# Autodesk Inventor assembly: Assembly1
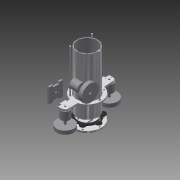
[picture p0: Inventor's stored thumbnail of the model, 180x180]
Saved by Autodesk Inventor 2015 (Build 190159000, 159)
## iProperties
Created: 2015-02-28
Part Number: Assembly1
Document SubType Name: Assembly
Designer: Qiuyang
Author: Qiuyang
## Documents named in this file (8)
- C:\Users\Qiuyang\Dropbox\VIP\SeaPerch\Dimensions\Aluminium_structure\Assembly1.iam
- C:\Users\Qiuyang\Dropbox\VIP\SeaPerch\Dimensions\Aluminium_structure\tube.ipt
- C:\Users\Qiuyang\Dropbox\VIP\SeaPerch\Dimensions\Aluminium_structure\rubber ring.ipt
- C:\Users\Qiuyang\Dropbox\VIP\SeaPerch\Dimensions\Aluminium_structure\threaded rod.ipt
- C:\Users\Qiuyang\Dropbox\VIP\SeaPerch\Dimensions\Aluminium_structure\cap with wire cut.ipt
- C:\Users\Qiuyang\Dropbox\VIP\SeaPerch\Dimensions\Aluminium_structure\middle plate.ipt
- C:\Users\Qiuyang\Dropbox\VIP\SeaPerch\Dimensions\Aluminium_structure\motor.ipt
- C:\Users\Qiuyang\Dropbox\VIP\SeaPerch\Dimensions\Aluminium_structure\motor holder.ipt
## Components (12 placed, 7 different names)
1. tube:1 — Insert:1, Insert:6, Insert:7
2. threaded rod:1 — Insert:5
3. threaded rod:2 — Insert:4
4. threaded rod:3 — Insert:3
5. rubber ring:1 — Insert:1, Insert:3, Insert:4, Insert:5
6. cap with wire cut:1 — Insert:6
7. middle plate:1 — Insert:7, Insert:8, Insert:9, Insert:10, Insert:11
8. motor:1 — Insert:8, Insert:11
9. motor:2 — Insert:9, Insert:10
10. motor:3
11. motor holder:1
12. motor holder:2
## Relationships (10: Insert 10)
- Insert:1 (12.7 mm): tube:1 ↔ rubber ring:1
- Insert:3 (6.35 mm): threaded rod:3 ↔ rubber ring:1
- Insert:4 (6.35 mm): threaded rod:2 ↔ rubber ring:1
- Insert:5 (6.35 mm): threaded rod:1 ↔ rubber ring:1
- Insert:6 (25.4 mm): tube:1 ↔ cap with wire cut:1
- Insert:7 (-152.4 mm): tube:1 ↔ middle plate:1
- Insert:8: middle plate:1 ↔ motor:1
- Insert:9: middle plate:1 ↔ motor:2
- Insert:10: middle plate:1 ↔ motor:2
- Insert:11: middle plate:1 ↔ motor:1
